# Autodesk Inventor assembly: Cube 1x1 V5 (Half Inch Lense)
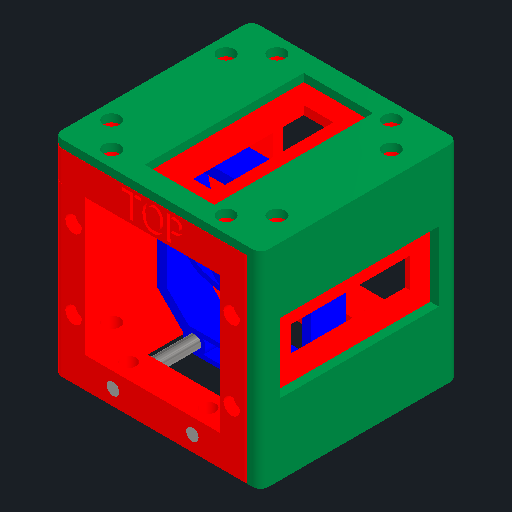
[picture p0: Inventor's stored thumbnail of the model, 512x512]
Saved by Autodesk Inventor 2023.4 (Build 274418000, 418)
## iProperties
Created: 2022-08-13
Part Number: Cube 1x1 V5 (Half Inch Lense)
Document SubType Name: Assembly
Designer: xSibe
Author: xSibe
## Documents named in this file (6)
- C:\.Laptop\.Work\Projects\Project Protocube\Protocube\CAD, STL, OBJ Files\1 CAD\Lens\Cube 1x1 V5 (Half Inch Lens).iam
- C:\.Laptop\.Work\Projects\Project Protocube\Protocube\CAD, STL, OBJ Files\1 CAD\Accessories\Mounting Bar.ipt
- C:\.Laptop\.Work\Projects\Project Protocube\Protocube\CAD, STL, OBJ Files\1 CAD\Lens\Half Inch Lens Mount (V5).ipt
- C:\.Laptop\.Work\Projects\Project Protocube\Protocube\CAD, STL, OBJ Files\1 CAD\Cubes\Cube 1x1 V5 Closed Slotted.iam
- C:\.Laptop\.Work\Projects\Project Protocube\Protocube\CAD, STL, OBJ Files\1 CAD\Lens\Half Inch Lens Mount Cover (V5).ipt
- C:\.Laptop\.Work\Projects\Project Protocube\Protocube\CAD, STL, OBJ Files\1 CAD\Covers\Outer Cover Open.ipt
## Components (5 placed, 5 different names)
1. Mounting Bar:1 — Mate:3, Mate:4
2. Half Inch Lens Mount (V5):1 — Mate:1, Mate:2, Mate:3, Mate:4, Flush:2
3. Cube 1x1 V5 Closed Slotted:1 [sub-assembly] — Mate:5, Mate:6, Mate:7
4. Half Inch Lens Mount Cover (V5):1 — Mate:1, Mate:2, Flush:1
5. Outer Cover Open:1 — Mate:5, Mate:6, Mate:7
## Relationships (9: Mate 7, Flush 2)
- Mate:1: Half Inch Lens Mount (V5):1 ↔ Half Inch Lens Mount Cover (V5):1
- Mate:2: Half Inch Lens Mount (V5):1 ↔ Half Inch Lens Mount Cover (V5):1
- Flush:1: Half Inch Lens Mount Cover (V5):1
- Mate:3: Mounting Bar:1 ↔ Half Inch Lens Mount (V5):1
- Mate:4: Mounting Bar:1 ↔ Half Inch Lens Mount (V5):1
- Flush:2: Half Inch Lens Mount (V5):1
- Mate:5: Cube 1x1 V5 Closed Slotted:1 ↔ Outer Cover Open:1
- Mate:6: Cube 1x1 V5 Closed Slotted:1 ↔ Outer Cover Open:1
- Mate:7: Cube 1x1 V5 Closed Slotted:1 ↔ Outer Cover Open:1
